# Autodesk Inventor assembly: sumoo
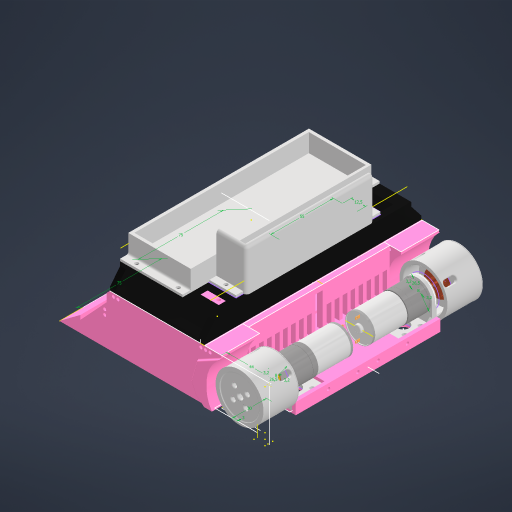
[picture p0: Inventor's stored thumbnail of the model, 512x512]
Saved by Autodesk Inventor 2024.3 (Build 283343000, 343)
## iProperties
Created: 2025-05-27
Part Number: sumoo
Document SubType Name: Assembly
Designer: Akbar Syihabuddin
Author: Akbar Syihabuddin
## Documents named in this file (11)
- C:\Users\GAMING 3i\OneDrive\Documents\desain inventor\sumo\sumoo.iam
- C:\Users\GAMING 3i\OneDrive\Documents\desain inventor\sumo\base.ipt
- C:\Users\GAMING 3i\OneDrive\Documents\desain inventor\sumo\blade.ipt
- C:\Users\GAMING 3i\OneDrive\Documents\desain inventor\sumo\hub 4mm.ipt
- C:\Users\GAMING 3i\OneDrive\Documents\desain inventor\sumo\jga25.ipt
- C:\Users\GAMING 3i\OneDrive\Documents\desain inventor\sumo\bracket bener.ipt
- C:\Users\GAMING 3i\OneDrive\Documents\desain inventor\sumo\bumper belakang.ipt
- C:\Users\GAMING 3i\OneDrive\Documents\desain inventor\sumo\roda.ipt
- C:\Users\GAMING 3i\OneDrive\Documents\desain inventor\sumo\atap.ipt
- C:\Users\GAMING 3i\OneDrive\Documents\desain inventor\sumo\beban.ipt
- C:\Users\GAMING 3i\OneDrive\Documents\desain inventor\sumo\batre.ipt
## Components (14 placed, 10 different names)
1. base:1 — Rigid:25, Rigid:26, Rigid:27, Rigid:28, Rigid:29
2. blade:1 — Rigid:25
3. hub 4mm:2 — Rotational:2, Rotational:3
4. hub 4mm:3 — Rotational:1, Rotational:4
5. jga25:1 — Rotational:2, Rigid:24
6. jga25:2 — Rotational:1, Rigid:23
7. bracket bener:1 — Rigid:23, Rigid:28
8. bracket bener:2 — Rigid:24, Rigid:26
9. bumper belakang:1 — Rigid:27
10. roda:1 — Rotational:4
11. roda:2 — Rotational:3
12. atap:1 — Rigid:29, Rigid:30, Rigid:31
13. beban:1 — Rigid:30
14. batre:1 — Rigid:31
## Relationships (13: WeldJoint 9, RevoluteJoint 4)
- Rotational:1 [RevoluteJoint]: hub 4mm:3 ↔ jga25:2
- Rotational:2 [RevoluteJoint]: hub 4mm:2 ↔ jga25:1
- Rigid:23 [WeldJoint]: jga25:2 ↔ bracket bener:1
- Rigid:24 [WeldJoint]: jga25:1 ↔ bracket bener:2
- Rigid:25 [WeldJoint]: base:1 ↔ blade:1
- Rigid:26 [WeldJoint]: base:1 ↔ bracket bener:2
- Rigid:27 [WeldJoint]: base:1 ↔ bumper belakang:1
- Rotational:3 [RevoluteJoint]: hub 4mm:2 ↔ roda:2
- Rotational:4 [RevoluteJoint]: hub 4mm:3 ↔ roda:1
- Rigid:28 [WeldJoint]: base:1 ↔ bracket bener:1
- Rigid:29 [WeldJoint]: base:1 ↔ atap:1
- Rigid:30 [WeldJoint]: atap:1 ↔ beban:1
- Rigid:31 [WeldJoint]: atap:1 ↔ batre:1
